# Autodesk Inventor assembly: 头洞四方轴套反装
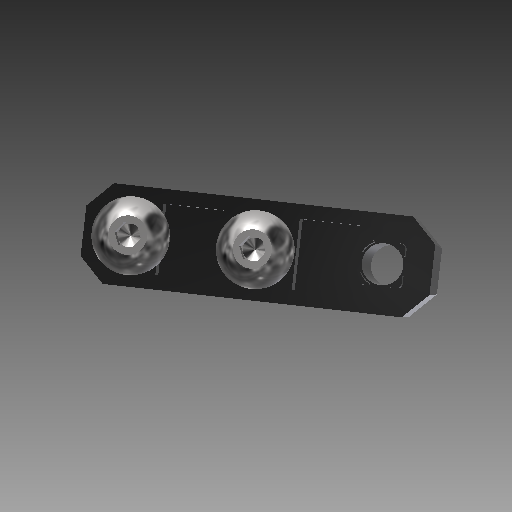
[picture p0: Inventor's stored thumbnail of the model, 512x512]
Saved by Autodesk Inventor 2019.3 (Build 233278000, 278)
## iProperties
Created: 2018-09-10
Part Number: 头洞四方轴套反装
Material: 常规
Document SubType Name: Assembly
Designer: aresp
Mass: 8.20296 g
Surface Area: 29.2574 cm^2
Volume: 2.34608 cm^3
Density: 3.49645 g/cm^3
Author: aresp
## Documents named in this file (4)
- D:\cad\零件库\头洞四方轴套反装.iam
- D:\cad\零件库\垫片轴套大白等\Bearing Flat.ipt
- D:\cad\零件库\螺丝螺帽\Screw 8-32 x 0.500'' - Black.ipt
- D:\cad\零件库\螺丝螺帽\Nut 8-32 Keps.ipt
## Components (5 placed, 3 different names)
1. Bearing Flat:1
2. Screw 8-32 x 0.500'' - Black:1
3. Screw 8-32 x 0.500'' - Black:2
4. Nut 8-32 Keps:1
5. Nut 8-32 Keps:2
## Relationships (2: Insert 2)
- [Insert]: Bearing Flat:1 ↔ Nut 8-32 Keps:1
- [Insert]: Bearing Flat:1 ↔ Nut 8-32 Keps:2
